# Autodesk Inventor assembly: 3A.01.08.JS.Rib 8
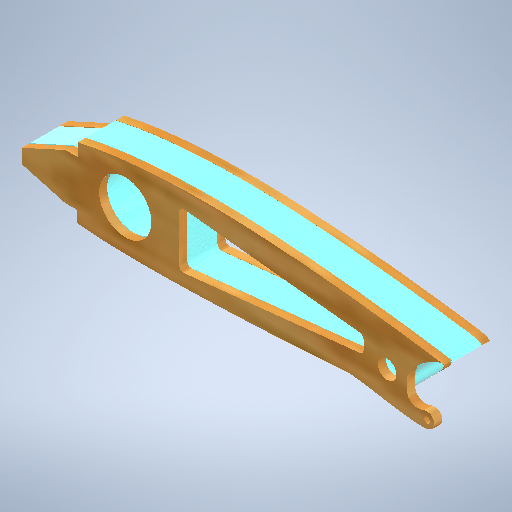
[picture p0: Inventor's stored thumbnail of the model, 512x512]
Saved by Autodesk Inventor 2025.1 (Build 291241000, 241)
## iProperties
Created: 2025-01-14
Part Number: 3A.01.08.JS.Rib 8
Document SubType Name: Assembly
Designer: johan
Mass: 22.4808 g
Surface Area: 456.482 cm^2
Volume: 104.546 cm^3
Density: 0.215033 g/cm^3
Author: johan
## Documents named in this file (4)
- C:\Users\chowg\OneDrive\Documents\Inventor\AVDASI 2 Group Project\assembly\3A.01.08.JS.Rib 8.iam
- C:\Users\chowg\OneDrive\Documents\Inventor\AVDASI 2 Group Project\assembly\3P.03.08.01.JS.rib 8 ply.ipt
- C:\Users\chowg\OneDrive\Documents\Inventor\AVDASI 2 Group Project\assembly\3P.03.08.02.JS.rib 8 foam.ipt
- C:\Users\chowg\OneDrive\Documents\Inventor\AVDASI 2 Group Project\assembly\3P.03.08.03.JS.rib 8 hinge ply.ipt
## Components (3 placed, 3 different names)
1. 3P.03.08.01.JS.rib 8 ply:1 — Rigid:1
2. 3P.03.08.02.JS.rib 8 foam:1 — Rigid:1, Rigid:2
3. 3P.03.08.03.JS.rib 8 hinge ply:1 — Rigid:2
## Relationships (2: WeldJoint 2)
- Rigid:1 [WeldJoint]: 3P.03.08.01.JS.rib 8 ply:1 ↔ 3P.03.08.02.JS.rib 8 foam:1
- Rigid:2 [WeldJoint]: 3P.03.08.02.JS.rib 8 foam:1 ↔ 3P.03.08.03.JS.rib 8 hinge ply:1
